# Autodesk Inventor assembly: ASSY_GB
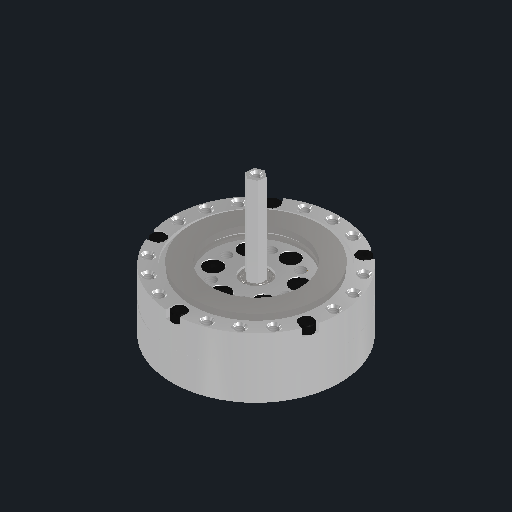
[picture p0: Inventor's stored thumbnail of the model, 512x512]
Saved by Autodesk Inventor 2024.2 (Build 282272000, 272)
## iProperties
Created: 2026-01-04
Part Number: ASSY_GB
Document SubType Name: Assembly
Designer: 4aida
Mass: 742.148 g
Surface Area: 1006.71 cm^2
Volume: 152.486 cm^3
Density: 4.86699 g/cm^3
Author: 4aida
## Documents named in this file (14)
- C:\Users\4aida\OneDrive\Documents\CADING\DESIGN FILES\6A-ROBO,BR6,2\GB\ASSY_GB.iam
- C:\Users\4aida\OneDrive\Documents\CADING\DESIGN FILES\6A-ROBO,BR6,2\GB\SHAFT_GB.ipt
- C:\Users\4aida\OneDrive\Documents\CADING\DESIGN FILES\6A-ROBO,BR6,2\GB\Case_GB.ipt
- C:\Users\4aida\OneDrive\Documents\CADING\DESIGN FILES\6A-ROBO,BR6,2\GB\Case_Taped_GB.ipt
- C:\Users\4aida\OneDrive\Documents\CADING\DESIGN FILES\Fasteners\M4\Hex Cap M4X20.ipt
- C:\Users\4aida\OneDrive\Documents\CADING\DESIGN FILES\6A-ROBO,BR6,2\GB\Thrust_Bearing-GB.ipt
- C:\Users\4aida\OneDrive\Documents\CADING\DESIGN FILES\6A-ROBO,BR6,2\GB\Case_Bearing_GB.ipt
- C:\Users\4aida\OneDrive\Documents\CADING\DESIGN FILES\6A-ROBO,BR6,2\GB\Cycloid_N20_E1_Rr2_R30.ipt
- C:\Users\4aida\OneDrive\Documents\CADING\DESIGN FILES\6A-ROBO,BR6,2\GB\Bearing_GB.ipt
- C:\Users\4aida\Downloads\1611-0514-4008\1611-0514-4008\1611-0514-4008.ipt
- C:\Users\4aida\OneDrive\Documents\CADING\DESIGN FILES\Fasteners\M4\DOWEL,M4X20.ipt
- C:\Users\4aida\OneDrive\Documents\CADING\DESIGN FILES\6A-ROBO,BR6,2\GB\Carier_Plate_GB.ipt
- C:\Users\4aida\OneDrive\Documents\CADING\DESIGN FILES\6A-ROBO,BR6,2\GB\Standoff_GB.ipt
- C:\Users\4aida\OneDrive\Documents\CADING\DESIGN FILES\Fasteners\M4\SCREW, FLAT HD, P, 12_9, M4X0_7X10MM.ipt
## Components (58 placed, 13 different names)
1. SHAFT_GB:1 — Mate:7, Mate:8, Flush:1, Flush:2
2. Case_GB:1 — Mate:15, Mate:16, Insert:21, Insert:22, Insert:23, Insert:24, Insert:25, Insert:26, Mate:42, Mate:44
3. Case_Taped_GB:1 — Mate:13, Mate:14, Insert:27, Mate:21, Mate:22, Mate:23, Mate:24, Mate:25, Mate:26, Mate:27, Mate:28, Mate:29, Mate:30, Mate:31, Mate:32, Mate:33, Mate:34, Mate:35, Mate:36, Mate:37, Mate:38, Mate:39, Mate:40, Mate:41, Mate:42, Mate:43, Mate:44
4. Hex Cap M4X20:1 — Insert:23
5. Hex Cap M4X20:2 — Insert:25
6. Hex Cap M4X20:3 — Insert:22
7. Hex Cap M4X20:4 — Insert:24, Mate:43
8. Hex Cap M4X20:5 — Insert:21
9. Thrust_Bearing-GB:1 — Mate:15, Mate:16
10. Thrust_Bearing-GB:2 — Mate:13, Mate:14
11. Case_Bearing_GB:1 — Insert:26
12. Case_Bearing_GB:2 — Insert:27, Mate:17, Mate:18
13. Cycloid_N20_E1_Rr2_R30:1 — Mate:9, Mate:11, Flush:3
14. Cycloid_N20_E1_Rr2_R30:2 — Mate:9, Mate:10, Mate:12, Mate:17
15. Bearing_GB:1 — Mate:8, Flush:1, Mate:10
16. Bearing_GB:2 — Mate:7, Flush:2, Mate:11, Flush:3
17. 1611-0514-4008:1 — Mate:5, Mate:6
18. 1611-0514-4008:2 — Mate:3, Mate:4
19. DOWEL,M4X20:1 — Mate:21, Mate:22, Flush:4, Flush:8, Flush:26
20. Carier_Plate_GB:1 — Mate:5, Mate:6
21. Carier_Plate_GB:2 — Mate:3, Mate:4, Mate:12, Mate:18
22. Standoff_GB:1
23. Standoff_GB:2
24. Standoff_GB:3
25. Standoff_GB:4
26. Standoff_GB:5
27. Standoff_GB:6
28. SCREW, FLAT HD, P, 12_9, M4X0_7X10MM:1
29. SCREW, FLAT HD, P, 12_9, M4X0_7X10MM:2
30. SCREW, FLAT HD, P, 12_9, M4X0_7X10MM:3
31. SCREW, FLAT HD, P, 12_9, M4X0_7X10MM:4
32. SCREW, FLAT HD, P, 12_9, M4X0_7X10MM:5
33. SCREW, FLAT HD, P, 12_9, M4X0_7X10MM:6
34. SCREW, FLAT HD, P, 12_9, M4X0_7X10MM:7
35. SCREW, FLAT HD, P, 12_9, M4X0_7X10MM:8
36. SCREW, FLAT HD, P, 12_9, M4X0_7X10MM:9
37. SCREW, FLAT HD, P, 12_9, M4X0_7X10MM:10
38. SCREW, FLAT HD, P, 12_9, M4X0_7X10MM:11
39. SCREW, FLAT HD, P, 12_9, M4X0_7X10MM:12
40. DOWEL,M4X20:2 — Flush:18, Flush:20, Flush:21, Flush:22, Flush:23, Mate:29, Flush:24
41. DOWEL,M4X20:3 — Mate:23, Flush:6
42. DOWEL,M4X20:4 — Flush:15, Mate:38
43. DOWEL,M4X20:5 — Flush:19, Mate:37
44. DOWEL,M4X20:6 — Mate:32, Flush:26
45. DOWEL,M4X20:7 — Flush:19, Mate:30, Flush:24, Flush:25
46. DOWEL,M4X20:8 — Flush:20, Mate:33
47. DOWEL,M4X20:9 — Flush:21, Mate:31
48. DOWEL,M4X20:10 — Flush:22, Mate:28
49. DOWEL,M4X20:11 — Flush:23, Mate:27
50. DOWEL,M4X20:12 — Flush:14, Mate:39
51. DOWEL,M4X20:13 — Flush:13, Mate:40
52. DOWEL,M4X20:14 — Mate:41, Flush:25
53. DOWEL,M4X20:16 — Flush:10, Flush:18, Mate:36
54. DOWEL,M4X20:17 — Flush:9, Mate:35
55. DOWEL,M4X20:18 — Flush:8, Flush:9, Flush:10, Flush:13, Flush:14, Flush:15, Mate:34
56. DOWEL,M4X20:19 — Mate:26, Flush:7
57. DOWEL,M4X20:20 — Mate:24, Flush:4, Flush:5, Flush:6
58. DOWEL,M4X20:21 — Mate:25, Flush:5, Flush:7
## Relationships (91: Mate 42, Insert 27, Flush 22)
- [Mate] (35 mm): 1611-0514-4008:1 ↔ DOWEL,M4X20:1
- [Insert]: Carier_Plate_GB:1 ↔ Standoff_GB:6
- [Insert]: Carier_Plate_GB:1 ↔ Standoff_GB:5
- [Insert]: Carier_Plate_GB:1 ↔ Standoff_GB:4
- [Insert]: Carier_Plate_GB:1 ↔ Standoff_GB:3
- [Insert]: Carier_Plate_GB:1 ↔ Standoff_GB:1
- [Insert]: Carier_Plate_GB:1 ↔ Standoff_GB:2
- [Insert]: Carier_Plate_GB:2 ↔ Standoff_GB:1
- [Insert]: Carier_Plate_GB:2 ↔ Standoff_GB:2
- [Mate]: 1611-0514-4008:2 ↔ Carier_Plate_GB:2
- [Insert]: Carier_Plate_GB:2 ↔ SCREW, FLAT HD, P, 12_9, M4X0_7X10MM:10
- [Insert]: Carier_Plate_GB:2 ↔ SCREW, FLAT HD, P, 12_9, M4X0_7X10MM:8
- [Insert]: Carier_Plate_GB:2 ↔ SCREW, FLAT HD, P, 12_9, M4X0_7X10MM:6
- [Insert]: Carier_Plate_GB:2 ↔ SCREW, FLAT HD, P, 12_9, M4X0_7X10MM:4
- [Insert]: Carier_Plate_GB:2 ↔ SCREW, FLAT HD, P, 12_9, M4X0_7X10MM:5
- [Insert]: Carier_Plate_GB:2 ↔ SCREW, FLAT HD, P, 12_9, M4X0_7X10MM:9
- [Insert]: Carier_Plate_GB:1 ↔ SCREW, FLAT HD, P, 12_9, M4X0_7X10MM:7
- [Insert]: Carier_Plate_GB:1 ↔ SCREW, FLAT HD, P, 12_9, M4X0_7X10MM:1
- [Insert]: Carier_Plate_GB:1 ↔ SCREW, FLAT HD, P, 12_9, M4X0_7X10MM:2
- [Insert]: Carier_Plate_GB:1 ↔ SCREW, FLAT HD, P, 12_9, M4X0_7X10MM:3
- [Insert]: Carier_Plate_GB:1 ↔ SCREW, FLAT HD, P, 12_9, M4X0_7X10MM:12
- [Insert]: Carier_Plate_GB:1 ↔ SCREW, FLAT HD, P, 12_9, M4X0_7X10MM:11
- Mate:3: 1611-0514-4008:2 ↔ Carier_Plate_GB:2
- Mate:4: 1611-0514-4008:2 ↔ Carier_Plate_GB:2
- Mate:5: 1611-0514-4008:1 ↔ Carier_Plate_GB:1
- Mate:6: 1611-0514-4008:1 ↔ Carier_Plate_GB:1
- Mate:7: SHAFT_GB:1 ↔ Bearing_GB:2
- Mate:8: SHAFT_GB:1 ↔ Bearing_GB:1
- Flush:1: SHAFT_GB:1 ↔ Bearing_GB:1
- Flush:2: SHAFT_GB:1 ↔ Bearing_GB:2
- Mate:9: Cycloid_N20_E1_Rr2_R30:1 ↔ Cycloid_N20_E1_Rr2_R30:2
- Mate:10: Cycloid_N20_E1_Rr2_R30:2 ↔ Bearing_GB:1
- Mate:11: Cycloid_N20_E1_Rr2_R30:1 ↔ Bearing_GB:2
- Mate:12: Cycloid_N20_E1_Rr2_R30:2 ↔ Carier_Plate_GB:2
- Mate:13: Case_Taped_GB:1 ↔ Thrust_Bearing-GB:2
- Mate:14: Case_Taped_GB:1 ↔ Thrust_Bearing-GB:2
- Mate:15: Case_GB:1 ↔ Thrust_Bearing-GB:1
- Mate:16: Case_GB:1 ↔ Thrust_Bearing-GB:1
- Insert:21: Case_GB:1 ↔ Hex Cap M4X20:5
- Insert:22: Case_GB:1 ↔ Hex Cap M4X20:3
- Insert:23: Case_GB:1 ↔ Hex Cap M4X20:1
- Insert:24: Case_GB:1 ↔ Hex Cap M4X20:4
- Insert:25: Case_GB:1 ↔ Hex Cap M4X20:2
- Insert:26: Case_GB:1 ↔ Case_Bearing_GB:1
- Insert:27: Case_Taped_GB:1 ↔ Case_Bearing_GB:2
- Mate:17: Case_Bearing_GB:2 ↔ Cycloid_N20_E1_Rr2_R30:2
- Flush:3: Cycloid_N20_E1_Rr2_R30:1 ↔ Bearing_GB:2
- Mate:18: Case_Bearing_GB:2 ↔ Carier_Plate_GB:2
- Mate:21: Case_Taped_GB:1 ↔ DOWEL,M4X20:1
- Mate:22: Case_Taped_GB:1 ↔ DOWEL,M4X20:1
- Mate:23: Case_Taped_GB:1 ↔ DOWEL,M4X20:3
- Mate:24: Case_Taped_GB:1 ↔ DOWEL,M4X20:20
- Mate:25: Case_Taped_GB:1 ↔ DOWEL,M4X20:21
- Mate:26: Case_Taped_GB:1 ↔ DOWEL,M4X20:19
- Flush:4: DOWEL,M4X20:1 ↔ DOWEL,M4X20:20
- Flush:5: DOWEL,M4X20:20 ↔ DOWEL,M4X20:21
- Flush:6: DOWEL,M4X20:3 ↔ DOWEL,M4X20:20
- Flush:7: DOWEL,M4X20:19 ↔ DOWEL,M4X20:21
- Flush:8: DOWEL,M4X20:1 ↔ DOWEL,M4X20:18
- Flush:9: DOWEL,M4X20:17 ↔ DOWEL,M4X20:18
- Flush:10: DOWEL,M4X20:16 ↔ DOWEL,M4X20:18
- Flush:13: DOWEL,M4X20:13 ↔ DOWEL,M4X20:18
- Flush:14: DOWEL,M4X20:12 ↔ DOWEL,M4X20:18
- Flush:15: DOWEL,M4X20:4 ↔ DOWEL,M4X20:18
- Flush:18: DOWEL,M4X20:2 ↔ DOWEL,M4X20:16
- Flush:19: DOWEL,M4X20:5 ↔ DOWEL,M4X20:7
- Flush:20: DOWEL,M4X20:2 ↔ DOWEL,M4X20:8
- Flush:21: DOWEL,M4X20:2 ↔ DOWEL,M4X20:9
- Flush:22: DOWEL,M4X20:2 ↔ DOWEL,M4X20:10
- Flush:23: DOWEL,M4X20:2 ↔ DOWEL,M4X20:11
- Mate:27: Case_Taped_GB:1 ↔ DOWEL,M4X20:11
- Mate:28: Case_Taped_GB:1 ↔ DOWEL,M4X20:10
- Mate:29: Case_Taped_GB:1 ↔ DOWEL,M4X20:2
- Mate:30: Case_Taped_GB:1 ↔ DOWEL,M4X20:7
- Mate:31: Case_Taped_GB:1 ↔ DOWEL,M4X20:9
- Mate:32: Case_Taped_GB:1 ↔ DOWEL,M4X20:6
- Mate:33: Case_Taped_GB:1 ↔ DOWEL,M4X20:8
- Mate:34: Case_Taped_GB:1 ↔ DOWEL,M4X20:18
- Mate:35: Case_Taped_GB:1 ↔ DOWEL,M4X20:17
- Mate:36: Case_Taped_GB:1 ↔ DOWEL,M4X20:16
- Mate:37: Case_Taped_GB:1 ↔ DOWEL,M4X20:5
- Mate:38: Case_Taped_GB:1 ↔ DOWEL,M4X20:4
- Mate:39: Case_Taped_GB:1 ↔ DOWEL,M4X20:12
- Mate:40: Case_Taped_GB:1 ↔ DOWEL,M4X20:13
- Mate:41: Case_Taped_GB:1 ↔ DOWEL,M4X20:14
- Flush:24: DOWEL,M4X20:2 ↔ DOWEL,M4X20:7
- Flush:25: DOWEL,M4X20:7 ↔ DOWEL,M4X20:14
- Flush:26: DOWEL,M4X20:1 ↔ DOWEL,M4X20:6
- Mate:42: Case_GB:1 ↔ Case_Taped_GB:1
- Mate:43: Case_Taped_GB:1 ↔ Hex Cap M4X20:4
- Mate:44: Case_GB:1 ↔ Case_Taped_GB:1
